# Autodesk Inventor assembly: MorotFixation_CounterWeightHolder_Assembly
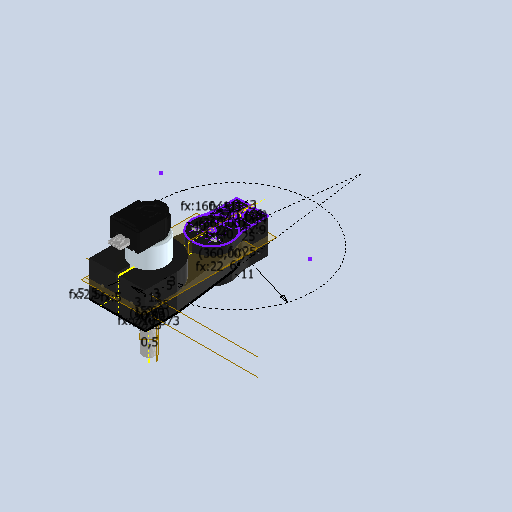
[picture p0: Inventor's stored thumbnail of the model, 512x512]
Saved by Autodesk Inventor 2024 (Build 280153000, 153)
## iProperties
Created: 2022-08-03
Part Number: MorotFixation_CounterWeightHolder_Assembly
Document SubType Name: Assembly
Designer: alexw
Mass: 623.224 g
Surface Area: 724.179 cm^2
Volume: 246.049 cm^3
Author: alexw
## Documents named in this file (9)
- C:\Users\AEWALDER\Documents\Inventor\03_CurrentProjects\MasterThesis\PSM_V1_Rillenkugellager\MorotFixation_CounterWeightHolder_Assembly.iam
- C:\Users\AEWALDER\Documents\Inventor\03_CurrentProjects\MasterThesis\PSM_V1_Rillenkugellager\ParallelMech_DrivenPart_Motor_GC_ShaftConnector.ipt
- C:\Users\AEWALDER\Documents\Inventor\03_CurrentProjects\MasterThesis\PSM_V1_Rillenkugellager\GC_Motor_Aussenscheibe.ipt
- C:\Users\AEWALDER\Documents\Inventor\03_CurrentProjects\MasterThesis\PSM_V1_Rillenkugellager\273752_RE35_GB_90W_KL_2WE.ipt
- C:\Users\AEWALDER\Documents\Inventor\03_CurrentProjects\MasterThesis\PSM_V1_Rillenkugellager\ContentCenter\de-DE\ISO 4762(2)\ISO 4762 - M5 x 50ISO.ipt
- C:\Users\AEWALDER\Documents\Inventor\03_CurrentProjects\MasterThesis\PSM_V1_Rillenkugellager\ContentCenter\de-DE\ISO 4762(2)\ISO 4762 - M4 x 30ISO.ipt
- C:\Users\AEWALDER\Documents\Inventor\03_CurrentProjects\MasterThesis\PSM_V1_Rillenkugellager\Shaft_6mmx36mm.ipt
- C:\Users\AEWALDER\Documents\Inventor\03_CurrentProjects\MasterThesis\PSM_V1_Rillenkugellager\AVAGO_HEDS_5540_A1.ipt
- C:\Users\AEWALDER\Documents\Inventor\03_CurrentProjects\MasterThesis\PSM_V1_Rillenkugellager\Capston_Drive_Motorwelle.ipt
## Components (10 placed, 8 different names)
1. ParallelMech_DrivenPart_Motor_GC_ShaftConnector:1 — Passend:1, Passend:2, Fluchtend:1, Passend:10, Passend:11, Passend:12, Passend:13, Passend:14, Fluchtend:2, Passend:20
2. GC_Motor_Aussenscheibe:1 — Passend:6, Passend:7, Passend:8, Passend:9, Passend:15, Fluchtend:3, Passend:18, Passend:19, Passend:20, Winkel:1
3. 273752_RE35_GB_90W_KL_2WE:1 — Passend:15, Fluchtend:3, Passend:21, Passend:22, Mate:23, Mate:24
4. ISO 4762 M5 x 50:1 — Passend:6, Passend:7
5. ISO 4762 M5 x 50:2 — Passend:8, Passend:9
6. ISO 4762 M4 x 30:1 — Passend:10, Passend:11
7. ISO 4762 M4 x 30:2 — Passend:12, Passend:13, Passend:19
8. Shaft_6mmx36mm:1 — Passend:14, Fluchtend:2, Passend:18
9. Capston_Drive_Motorwelle:1 — Mate:23, Mate:24
10. AVAGO_HEDS_5540_A1:1 — Passend:21, Winkel:1, Passend:22
## Relationships (23: Mate 19, Flush 3, Angle 1)
- Passend:1 [Mate]: ParallelMech_DrivenPart_Motor_GC_ShaftConnector:1
- Passend:2 [Mate]: ParallelMech_DrivenPart_Motor_GC_ShaftConnector:1
- Fluchtend:1 [Flush]: ParallelMech_DrivenPart_Motor_GC_ShaftConnector:1
- Passend:6 [Mate]: GC_Motor_Aussenscheibe:1 ↔ ISO 4762 M5 x 50:1
- Passend:7 [Mate]: GC_Motor_Aussenscheibe:1 ↔ ISO 4762 M5 x 50:1
- Passend:8 [Mate]: GC_Motor_Aussenscheibe:1 ↔ ISO 4762 M5 x 50:2
- Passend:9 [Mate]: GC_Motor_Aussenscheibe:1 ↔ ISO 4762 M5 x 50:2
- Passend:10 [Mate]: ParallelMech_DrivenPart_Motor_GC_ShaftConnector:1 ↔ ISO 4762 M4 x 30:1
- Passend:11 [Mate]: ParallelMech_DrivenPart_Motor_GC_ShaftConnector:1 ↔ ISO 4762 M4 x 30:1
- Passend:12 [Mate]: ParallelMech_DrivenPart_Motor_GC_ShaftConnector:1 ↔ ISO 4762 M4 x 30:2
- Passend:13 [Mate]: ParallelMech_DrivenPart_Motor_GC_ShaftConnector:1 ↔ ISO 4762 M4 x 30:2
- Passend:14 [Mate]: ParallelMech_DrivenPart_Motor_GC_ShaftConnector:1 ↔ Shaft_6mmx36mm:1
- Fluchtend:2 [Flush]: ParallelMech_DrivenPart_Motor_GC_ShaftConnector:1 ↔ Shaft_6mmx36mm:1
- Passend:15 [Mate]: GC_Motor_Aussenscheibe:1 ↔ 273752_RE35_GB_90W_KL_2WE:1
- Fluchtend:3 [Flush] (-13 mm): GC_Motor_Aussenscheibe:1 ↔ 273752_RE35_GB_90W_KL_2WE:1
- Passend:18 [Mate]: GC_Motor_Aussenscheibe:1 ↔ Shaft_6mmx36mm:1
- Passend:19 [Mate]: GC_Motor_Aussenscheibe:1 ↔ ISO 4762 M4 x 30:2
- Passend:20 [Mate]: ParallelMech_DrivenPart_Motor_GC_ShaftConnector:1 ↔ GC_Motor_Aussenscheibe:1
- Passend:21 [Mate]: 273752_RE35_GB_90W_KL_2WE:1 ↔ AVAGO_HEDS_5540_A1:1
- Winkel:1 [Angle] (0 deg): GC_Motor_Aussenscheibe:1 ↔ AVAGO_HEDS_5540_A1:1
- Passend:22 [Mate]: 273752_RE35_GB_90W_KL_2WE:1 ↔ AVAGO_HEDS_5540_A1:1
- Mate:23: 273752_RE35_GB_90W_KL_2WE:1 ↔ Capston_Drive_Motorwelle:1
- Mate:24: 273752_RE35_GB_90W_KL_2WE:1 ↔ Capston_Drive_Motorwelle:1
